# Autodesk Inventor assembly: Top_Beam
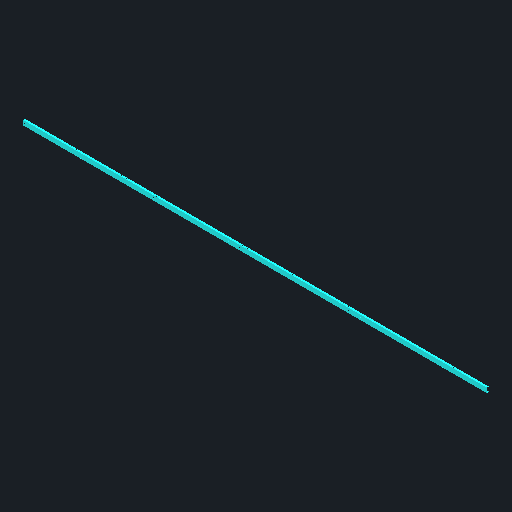
[picture p0: Inventor's stored thumbnail of the model, 512x512]
Saved by Autodesk Inventor 2025.3 (Build 293356030, 356C)
## iProperties
Created: 2019-12-15
Part Number: Top_Beam
Document SubType Name: Assembly
Designer: Rubens
Sending System: SolidWorks 2018
Last Author: Mohsen
Last Saved: 2022-08-25
Author: Rubens
## Documents named in this file (4)
- C:\Users\Rubens\Downloads\Estrutura Placa - REV00\Solar Mounting Structure\Main_Solar_Structure\Main_Solar_Structure\Top_Beam.iam
- C:\Users\Rubens\Downloads\Estrutura Placa - REV00\Solar Mounting Structure\Main_Solar_Structure\Main_Solar_Structure\Top_Beam_2780.ipt
- C:\Users\Rubens\Downloads\Estrutura Placa - REV00\Solar Mounting Structure\Main_Solar_Structure\Main_Solar_Structure\Top_Beam_2760.ipt
- C:\Users\Rubens\Downloads\Estrutura Placa - REV00\Solar Mounting Structure\Main_Solar_Structure\Main_Solar_Structure\Top_Beam_2770.ipt
## Components (3 placed, 3 different names)
1. Top_Beam_2780:1 — Alinhado:2, Coincidente:3, Coincidente:4
2. Top_Beam_2760:1 — Coincidente:1, Coincidente:2, Alinhado:1, Alinhado:2, Coincidente:3, Coincidente:4, Alinhado:3
3. Top_Beam_2770:1 — Coincidente:1, Coincidente:2, Alinhado:1, Alinhado:3
## Relationships (7: Mate 4, Flush 3)
- Coincidente:1 [Mate]: Top_Beam_2760:1 ↔ Top_Beam_2770:1
- Coincidente:2 [Mate]: Top_Beam_2760:1 ↔ Top_Beam_2770:1
- Alinhado:1 [Flush]: Top_Beam_2760:1 ↔ Top_Beam_2770:1
- Alinhado:2 [Flush]: Top_Beam_2780:1 ↔ Top_Beam_2760:1
- Coincidente:3 [Mate]: Top_Beam_2780:1 ↔ Top_Beam_2760:1
- Coincidente:4 [Mate]: Top_Beam_2780:1 ↔ Top_Beam_2760:1
- Alinhado:3 [Flush]: Top_Beam_2760:1 ↔ Top_Beam_2770:1
